# Autodesk Inventor assembly: TheCameraAssy-NEW
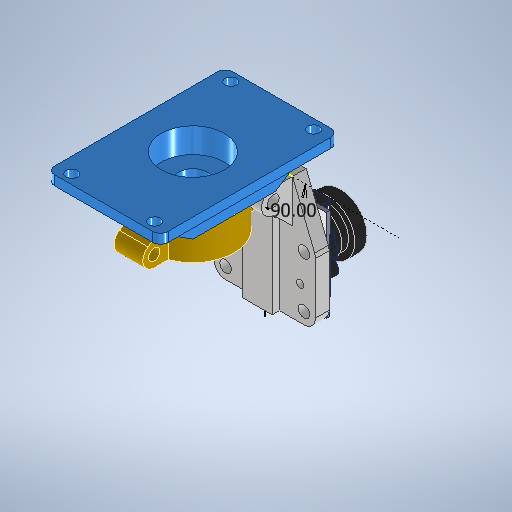
[picture p0: Inventor's stored thumbnail of the model, 512x512]
Saved by Autodesk Inventor 2025.1 (Build 291241000, 241)
## iProperties
Created: 2026-05-18
Part Number: TheCameraAssy-NEW
Document SubType Name: Assembly
Designer: User
Author: User
## Documents named in this file (5)
- D:\One Drive\OneDrive - Politeknik Sultan Salahuddin Abdul Aziz Shah\Documents\Inventor\RobosotPSA\TheCameraAssy-NEW.iam
- D:\One Drive\OneDrive - Politeknik Sultan Salahuddin Abdul Aziz Shah\Documents\Inventor\RobosotPSA\cameraholder_v3.ipt
- D:\One Drive\OneDrive - Politeknik Sultan Salahuddin Abdul Aziz Shah\Documents\Inventor\RobosotPSA\NewCameraHolder.ipt
- D:\One Drive\OneDrive - Politeknik Sultan Salahuddin Abdul Aziz Shah\Documents\Inventor\RobosotPSA\TheCamera.ipt
- D:\One Drive\OneDrive - Politeknik Sultan Salahuddin Abdul Aziz Shah\Documents\Inventor\RobosotPSA\rpiCameraMAssembly\rpiCameraMAssembly\rpiCameraMAssembly.ipt
## Components (4 placed, 4 different names)
1. cameraholder_v3:1 — Flush:1
2. NewCameraHolder:1 — Flush:1, Flush:2
3. TheCamera:1 — Flush:2
4. rpiCameraMAssembly:1
## Relationships (2: Flush 2)
- Flush:1: cameraholder_v3:1 ↔ NewCameraHolder:1
- Flush:2: NewCameraHolder:1 ↔ TheCamera:1
